# Autodesk Inventor assembly: WormDrive02
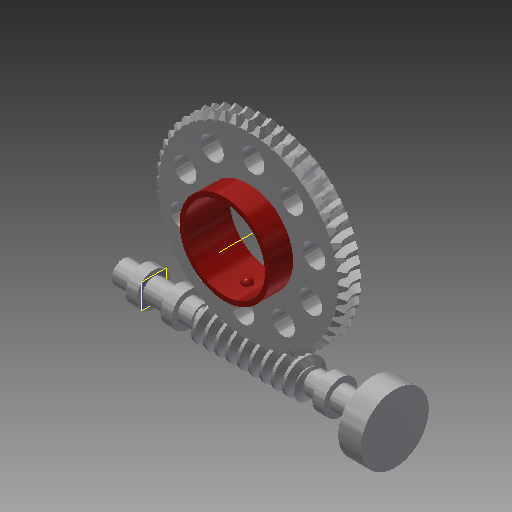
[picture p0: Inventor's stored thumbnail of the model, 512x512]
Saved by Autodesk Inventor 2019.3 (Build 233278000, 278)
## iProperties
Created: 2019-01-18
Part Number: WormDrive02
Document SubType Name: Assembly
Designer: steele
Author: steele
## Documents named in this file (3)
- C:\git\CAD-Development\robSteele\ShapeWays\TelescopeProjects\Focuser\WormDrive02.iam
- C:\git\CAD-Development\robSteele\ShapeWays\TelescopeProjects\Focuser\WormDrive02\Design Accelerator\Worm Gears1.iam
- C:\git\CAD-Development\robSteele\ShapeWays\TelescopeProjects\Focuser\ExternalMotorizedOuterRing.ipt
## Components (2 placed, 2 different names)
1. Worm Gears:1 [sub-assembly] — Angle:1, Mate:1, Mate:2
2. ExternalMotorizedOuterRing:1 — Mate:1, Mate:2
## Relationships (3: Mate 2, Angle 1)
- Angle:1 (0 deg): Worm Gears:1
- Mate:1 (6.5532 mm): Worm Gears:1 ↔ ExternalMotorizedOuterRing:1
- Mate:2: Worm Gears:1 ↔ ExternalMotorizedOuterRing:1
